# Autodesk Inventor assembly: Chain Drive5_MIR
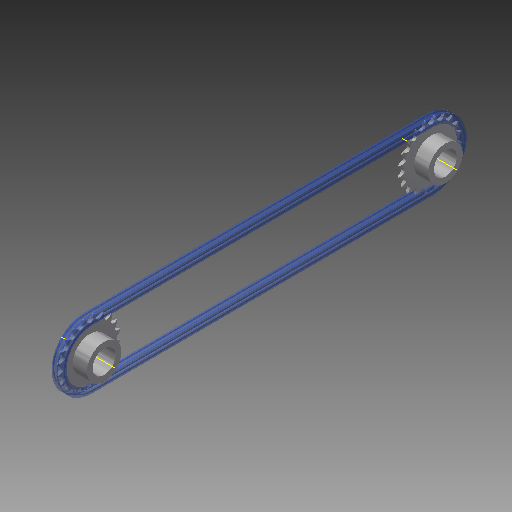
[picture p0: Inventor's stored thumbnail of the model, 512x512]
Saved by Autodesk Inventor 2019.4 (Build 234330000, 330)
## iProperties
Created: 2019-12-07
Part Number: Chain Drive5_MIR
Document SubType Name: Assembly
Designer: admin
Mass: 176.342 g
Surface Area: 386.546 cm^2
Volume: 50.2694 cm^3
Density: 3.50794 g/cm^3
Author: admin
## Documents named in this file (4)
- C:\Users\admin\Desktop\FRC 2020 Engineering\GitHub\7738-CAD-prep\WCD\WCD V2\Design Accelerator\Chain Drive5_MIR.iam
- C:\Users\admin\Desktop\FRC 2020 Engineering\GitHub\7738-CAD-prep\WCD\WCD V2\Design Accelerator\Roller Chain5_MIR.ipt
- C:\Users\admin\Desktop\FRC 2020 Engineering\GitHub\7738-CAD-prep\WCD\WCD V2\Design Accelerator\Roller Chain Sprocket14_MIR.ipt
- C:\Users\admin\Desktop\FRC 2020 Engineering\GitHub\7738-CAD-prep\WCD\WCD V2\Design Accelerator\Roller Chain Sprocket25_MIR.ipt
## Components (3 placed, 3 different names)
1. Roller Chain5_MIR:1 — Mate:2, Mate:1, Flush:1, Mate:4, Mate:3, Flush:2
2. Roller Chain Sprocket14_MIR:1 — Mate:2, Mate:1, Flush:1, Rotation:1
3. Roller Chain Sprocket25_MIR:1 — Mate:4, Mate:3, Flush:2, Rotation:1
## Relationships (7: Mate 4, Flush 2, RelateRotation 1)
- Mate:2: Roller Chain5_MIR:1 ↔ Roller Chain Sprocket14_MIR:1
- Mate:1: Roller Chain5_MIR:1 ↔ Roller Chain Sprocket14_MIR:1
- Flush:1: Roller Chain5_MIR:1 ↔ Roller Chain Sprocket14_MIR:1
- Mate:4: Roller Chain5_MIR:1 ↔ Roller Chain Sprocket25_MIR:1
- Mate:3: Roller Chain5_MIR:1 ↔ Roller Chain Sprocket25_MIR:1
- Flush:2: Roller Chain5_MIR:1 ↔ Roller Chain Sprocket25_MIR:1
- Rotation:1 [RelateRotation] (1 ul): Roller Chain Sprocket14_MIR:1 ↔ Roller Chain Sprocket25_MIR:1
